# Autodesk Inventor assembly: Stool Assembly
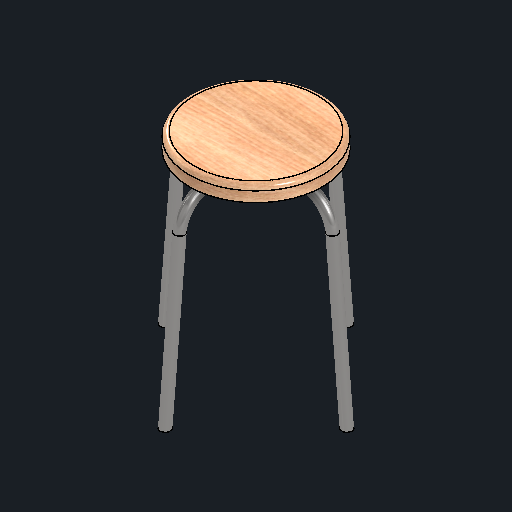
[picture p0: Inventor's stored thumbnail of the model, 512x512]
Saved by Autodesk Inventor 2026.2 (Build 302298000, 298)
## iProperties
Created: 2026-10-01
Part Number: Stool Assembly
Document SubType Name: Assembly
Designer: Joshua Eah
Author: Joshua Eah
## Documents named in this file (11)
- C:\Users\Joshua Eah\Documents\GitHub\designs\CFA Stool\Stool Assembly.iam
- C:\Users\Joshua Eah\Documents\GitHub\designs\CFA Stool\Seat.ipt
- C:\Users\Joshua Eah\Documents\GitHub\designs\CFA Stool\Leg.ipt
- C:\Users\Joshua Eah\Documents\GitHub\designs\CFA Stool\Pipe Adapter.ipt
- C:\Users\Joshua Eah\Documents\GitHub\designs\CFA Stool\No12x1.75 FH WD Screw.ipt
- C:\Users\Joshua Eah\Documents\GitHub\designs\CFA Stool\Stool Assembly\AIP\FEA\fki1hp83k.fins
- C:\Users\Joshua Eah\Documents\GitHub\designs\CFA Stool\Stool Assembly\AIP\FEA\fki1hp83k.fsat
- C:\Users\Joshua Eah\Documents\GitHub\designs\CFA Stool\Stool Assembly\AIP\FEA\fki1hp83k.ftes
- C:\Users\Joshua Eah\Documents\GitHub\designs\CFA Stool\Stool Assembly\AIP\FEA\fki1hp83k.fwiz
- C:\Users\Joshua Eah\Documents\GitHub\designs\CFA Stool\Stool Assembly\AIP\FEA\fki1hp880.fmsh
- C:\Users\Joshua Eah\Documents\GitHub\designs\CFA Stool\Stool Assembly\AIP\FEA\fki1hp881.fres
## Components (17 placed, 4 different names)
1. Seat:1 — Insert:1, Insert:2
2. Pipe Adapter:1 — Insert:1, Insert:2, Mate:1, Mate:2
3. Leg:1 — Mate:1, Mate:2, Mate:3, Transitional:1
4. Pipe Adapter:2
5. Leg:2
6. Pipe Adapter:3
7. Leg:3
8. Pipe Adapter:4
9. Leg:4
10. No12x1.75 FH WD Screw:1 — Mate:3, Transitional:1
11. No12x1.75 FH WD Screw:2
12. No12x1.75 FH WD Screw:3
13. No12x1.75 FH WD Screw:4
14. No12x1.75 FH WD Screw:5
15. No12x1.75 FH WD Screw:6
16. No12x1.75 FH WD Screw:7
17. No12x1.75 FH WD Screw:8
## Component patterns: (4 elements, first: Pipe Adapter:1 + Leg:1), (2 elements, first: No12x1.75 FH WD Screw:1), Component Pattern 8:2 (2 elements), Component Pattern 8:3 (2 elements), Component Pattern 8:4 (2 elements)
## Relationships (6: Mate 3, Insert 2, Transitional 1)
- Insert:1: Seat:1 ↔ Pipe Adapter:1
- Insert:2: Seat:1 ↔ Pipe Adapter:1
- Mate:1: Pipe Adapter:1 ↔ Leg:1
- Mate:2: Pipe Adapter:1 ↔ Leg:1
- Mate:3: Leg:1 ↔ No12x1.75 FH WD Screw:1
- Transitional:1: Leg:1 ↔ No12x1.75 FH WD Screw:1
## Named parameters: sa_0 = 88964.4
note: some values were not read from the file. Shown as the stored number, unit unknown: "sa_0".
